# Autodesk Inventor assembly: Ensamble_completo
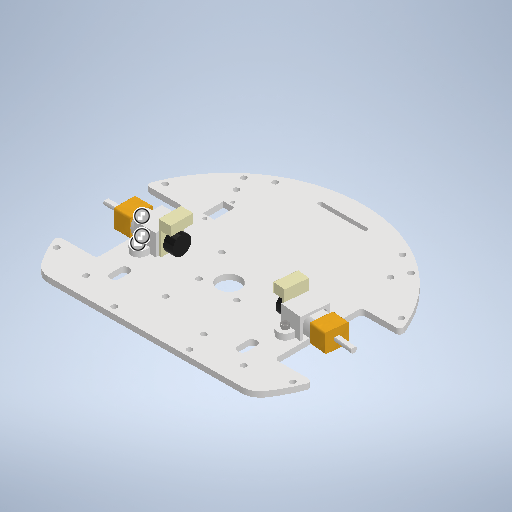
[picture p0: Inventor's stored thumbnail of the model, 512x512]
Saved by Autodesk Inventor 2025.3 (Build 293356030, 356C)
## iProperties
Created: 2025-10-21
Part Number: Ensamble_completo
Document SubType Name: Assembly
Designer: brene
Author: brene
## Documents named in this file (7)
- D:\OneDrive - Estudiantes ITCR\Documentos\GitHub\Atta-Bot-STEM\Chasis\Rediseño_Diego&Carlos\Carcasa 4.0 Rediseño\Ensamble_completo.iam
- D:\OneDrive - Estudiantes ITCR\Documentos\GitHub\Atta-Bot-STEM\Chasis\Rediseño_Diego&Carlos\Carcasa 4.0 Rediseño\base_chasis_v6\base_chasis_v4-dimsAjustadas.ipt
- D:\OneDrive - Estudiantes ITCR\Documentos\GitHub\Atta-Bot-STEM\Chasis\Rediseño_Diego&Carlos\Carcasa 4.0 Rediseño\base_chasis_v6.ipt
- D:\OneDrive - Estudiantes ITCR\Documentos\GitHub\Atta-Bot-STEM\Chasis\Rediseño_Diego&Carlos\motor.ipt
- D:\OneDrive - Estudiantes ITCR\Documentos\GitHub\Atta-Bot-STEM\Chasis\Rediseño_Diego&Carlos\soporteMotor_MIR.ipt
- D:\OneDrive - Estudiantes ITCR\Documentos\GitHub\Atta-Bot-STEM\Chasis\Rediseño_Diego&Carlos\Content Center Files\en-US\ISO 4762(2)\ISO 4762 - M2 x 8ISO.ipt
- D:\OneDrive - Estudiantes ITCR\Documentos\GitHub\Atta-Bot-STEM\Chasis\Rediseño_Diego&Carlos\Content Center Files\en-US\ISO 4032(2)\ISO 4032 - M2 - ISO.ipt
## Components (13 placed, 5 different names)
1. base_chasis_v4-dimsAjustadas:1 — Mate:1, Mate:2, Mate:3, Mate:5, Mate:6, Mate:7, Insert:2
2. motor:1 — Mate:7, Mate:8, Tangent:2
3. motor:2 — Mate:3, Mate:4, Tangent:1
4. soporteMotor_MIR:1 — Mate:5, Mate:6, Mate:8, Tangent:2, Mate:9, Insert:1, Mate:10, Insert:3
5. soporteMotor_MIR:2 — Mate:1, Mate:2, Mate:4, Tangent:1, Mate:11, Insert:5, Mate:12, Insert:6
6. ISO 4762 M2 x 8:1 — Mate:10, Insert:3, Insert:4
7. ISO 4762 M2 x 8:2 — Mate:9, Insert:1
8. ISO 4762 M2 x 8:3 — Mate:11, Insert:5, Insert:7
9. ISO 4762 M2 x 8:4 — Mate:12, Insert:6, Insert:8
10. ISO 4032 M2:1 — Insert:7
11. ISO 4032 M2:2 — Insert:8
12. ISO 4032 M2:3 — Insert:4
13. ISO 4032 M2:4 — Insert:2
## Relationships (22: Mate 12, Insert 8, Tangent 2)
- Mate:1: base_chasis_v4-dimsAjustadas:1 ↔ soporteMotor_MIR:2
- Mate:2: base_chasis_v4-dimsAjustadas:1 ↔ soporteMotor_MIR:2
- Mate:3: base_chasis_v4-dimsAjustadas:1 ↔ motor:2
- Mate:4: motor:2 ↔ soporteMotor_MIR:2
- Tangent:1: motor:2 ↔ soporteMotor_MIR:2
- Mate:5: base_chasis_v4-dimsAjustadas:1 ↔ soporteMotor_MIR:1
- Mate:6: base_chasis_v4-dimsAjustadas:1 ↔ soporteMotor_MIR:1
- Mate:7: base_chasis_v4-dimsAjustadas:1 ↔ motor:1
- Mate:8: motor:1 ↔ soporteMotor_MIR:1
- Tangent:2: motor:1 ↔ soporteMotor_MIR:1
- Mate:9: soporteMotor_MIR:1 ↔ ISO 4762 M2 x 8:2
- Insert:1: soporteMotor_MIR:1 ↔ ISO 4762 M2 x 8:2
- Insert:2: base_chasis_v4-dimsAjustadas:1 ↔ ISO 4032 M2:4
- Mate:10: soporteMotor_MIR:1 ↔ ISO 4762 M2 x 8:1
- Insert:3: soporteMotor_MIR:1 ↔ ISO 4762 M2 x 8:1
- Insert:4: ISO 4762 M2 x 8:1 ↔ ISO 4032 M2:3
- Mate:11: soporteMotor_MIR:2 ↔ ISO 4762 M2 x 8:3
- Insert:5: soporteMotor_MIR:2 ↔ ISO 4762 M2 x 8:3
- Mate:12: soporteMotor_MIR:2 ↔ ISO 4762 M2 x 8:4
- Insert:6: soporteMotor_MIR:2 ↔ ISO 4762 M2 x 8:4
- Insert:7: ISO 4762 M2 x 8:3 ↔ ISO 4032 M2:1
- Insert:8: ISO 4762 M2 x 8:4 ↔ ISO 4032 M2:2
